# Autodesk Inventor assembly: Ensamblaje1
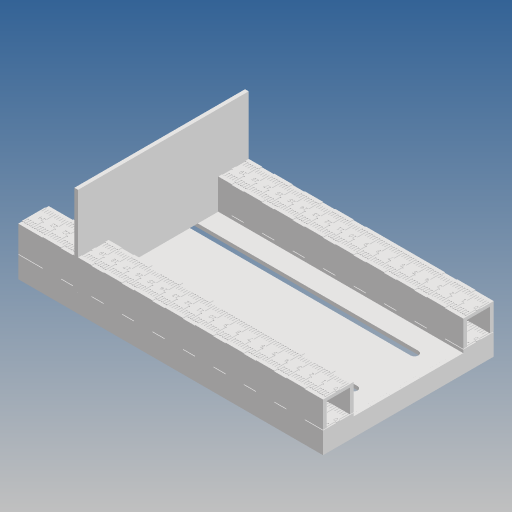
[picture p0: Inventor's stored thumbnail of the model, 512x512]
Saved by Autodesk Inventor 2024 (Build 280153000, 153)
## iProperties
Created: 2024-05-31
Part Number: Ensamblaje1
Document SubType Name: Assembly
Designer: Pablo
Author: Pablo
## Documents named in this file (7)
- D:\Users\Pablo\Desktop\UVG\otros\TesisM\Ensamblaje1.iam
- D:\Users\Pablo\Desktop\UVG\otros\TesisM\Pieza1.ipt
- D:\Users\Pablo\Desktop\UVG\otros\TesisM\Pieza2.ipt
- D:\Users\Pablo\Desktop\UVG\otros\TesisM\Pieza3.ipt
- D:\Users\Pablo\Desktop\UVG\otros\TesisM\Ensamblaje2.iam
- D:\Users\Pablo\Desktop\UVG\otros\TesisM\Ensamblaje3.iam
- D:\Users\Pablo\Desktop\UVG\otros\TesisM\Pieza10.ipt
## Components (9 placed, 6 different names)
1. Pieza1:1 — Coincidencia:1, Nivelación:3, Coincidencia:2, Nivelación:4, Nivelación:5, Nivelación:6, Nivelación:8, Coincidencia:3, Nivelación:14, Coincidencia:7, Coincidencia:8, Coincidencia:9, Coincidencia:12, Coincidencia:13, Coincidencia:14
2. Pieza2:1 — Coincidencia:1, Nivelación:5, Nivelación:7, Nivelación:9, Nivelación:14, Nivelación:17
3. Pieza2:2 — Nivelación:3, Coincidencia:2, Nivelación:4, Nivelación:18
4. Pieza3:1 — Nivelación:8, Nivelación:9, Coincidencia:3, Nivelación:15, Nivelación:16
5. Pieza3:2 — Nivelación:6, Nivelación:7, Coincidencia:8
6. Ensamblaje3:1 [sub-assembly] — Coincidencia:7, Coincidencia:9, Coincidencia:11
7. Pieza10:1 — Coincidencia:11, Coincidencia:12, Nivelación:19
8. Ensamblaje2:1 [sub-assembly] — Nivelación:16, Coincidencia:13, Nivelación:18
9. Ensamblaje2:2 [sub-assembly] — Nivelación:15, Coincidencia:14, Nivelación:17, Nivelación:19
## Relationships (23: Flush 13, Mate 10)
- Coincidencia:1 [Mate]: Pieza1:1 ↔ Pieza2:1
- Nivelación:3 [Flush]: Pieza1:1 ↔ Pieza2:2
- Coincidencia:2 [Mate]: Pieza1:1 ↔ Pieza2:2
- Nivelación:4 [Flush]: Pieza1:1 ↔ Pieza2:2
- Nivelación:5 [Flush]: Pieza1:1 ↔ Pieza2:1
- Nivelación:6 [Flush]: Pieza1:1 ↔ Pieza3:2
- Nivelación:7 [Flush]: Pieza2:1 ↔ Pieza3:2
- Nivelación:8 [Flush]: Pieza1:1 ↔ Pieza3:1
- Nivelación:9 [Flush]: Pieza2:1 ↔ Pieza3:1
- Coincidencia:3 [Mate]: Pieza1:1 ↔ Pieza3:1
- Nivelación:14 [Flush]: Pieza1:1 ↔ Pieza2:1
- Coincidencia:7 [Mate]: Pieza1:1 ↔ Ensamblaje3:1
- Coincidencia:8 [Mate]: Pieza1:1 ↔ Pieza3:2
- Coincidencia:9 [Mate]: Pieza1:1 ↔ Ensamblaje3:1
- Coincidencia:11 [Mate]: Ensamblaje3:1 ↔ Pieza10:1
- Coincidencia:12 [Mate]: Pieza1:1 ↔ Pieza10:1
- Nivelación:15 [Flush]: Pieza3:1 ↔ Ensamblaje2:2
- Nivelación:16 [Flush]: Pieza3:1 ↔ Ensamblaje2:1
- Coincidencia:13 [Mate]: Pieza1:1 ↔ Ensamblaje2:1
- Coincidencia:14 [Mate]: Pieza1:1 ↔ Ensamblaje2:2
- Nivelación:17 [Flush]: Pieza2:1 ↔ Ensamblaje2:2
- Nivelación:18 [Flush]: Pieza2:2 ↔ Ensamblaje2:1
- Nivelación:19 [Flush]: Pieza10:1 ↔ Ensamblaje2:2
